# Autodesk Inventor assembly: Stewart_Platform
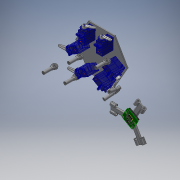
[picture p0: Inventor's stored thumbnail of the model, 180x180]
Saved by Autodesk Inventor 2019.4 (Build 234330000, 330)
## iProperties
Created: 2020-04-07
Part Number: Stewart_Platform
Document SubType Name: Assembly
Designer: Jorian Brusind
Author: Jorian Brusind
## Documents named in this file (7)
- C:\Users\Jorian Brusind\Documents\GitHub\PersonalProjects\Stewart Platform\Inventor Models\Stewart_Platform.iam
- C:\Users\Jorian Brusind\Documents\GitHub\PersonalProjects\Stewart Platform\Inventor Models\Top_.ipt
- C:\Users\Jorian Brusind\Documents\GitHub\PersonalProjects\Stewart Platform\Inventor Models\raspberry-pi-camera-module-v2-1.snapshot.3\RspCameraMia.iam
- C:\Users\Jorian Brusind\Documents\GitHub\PersonalProjects\Stewart Platform\Inventor Models\Bot_.ipt
- C:\Users\Jorian Brusind\Documents\GitHub\PersonalProjects\Stewart Platform\Inventor Models\tower-pro-sg90-micro-servo-2.snapshot.5\microservoAssembly.iam
- C:\Users\Jorian Brusind\Documents\GitHub\PersonalProjects\Stewart Platform\Inventor Models\tower-pro-sg90-micro-servo-2.snapshot.5\microservoArm.ipt
- C:\Users\Jorian Brusind\Documents\GitHub\PersonalProjects\Stewart Platform\Inventor Models\59935K140_METRIC BALL JOINT ROD END.ipt
## Components (21 placed, 6 different names)
1. Top_:1 — Mate:1, Mate:2, Mate:3
2. RspCameraMia:1 [sub-assembly] — Mate:1, Mate:2, Mate:3
3. Bot_:1 — Mate:4, Mate:5, Mate:6, Mate:7, Mate:8, Mate:9, Mate:10, Mate:11, Mate:12, Mate:13, Mate:14, Mate:15, Mate:16, Mate:17, Mate:18, Mate:19, Mate:20, Mate:21
4. microservoAssembly:1 [sub-assembly] — Mate:4, Mate:5, Mate:6, Mate:24, Mate:25
5. microservoAssembly:2 [sub-assembly] — Mate:8, Mate:9, Mate:10, Mate:22, Mate:23
6. microservoAssembly:3 [sub-assembly] — Mate:16, Mate:18, Mate:19, Mate:26, Mate:33
7. microservoAssembly:4 [sub-assembly] — Mate:11, Mate:12, Mate:13, Mate:29, Mate:31
8. microservoAssembly:5 [sub-assembly] — Mate:7, Mate:14, Mate:15, Mate:28, Mate:30
9. microservoAssembly:6 [sub-assembly] — Mate:17, Mate:20, Mate:21, Mate:27, Mate:32
10. microservoArm:1 — Mate:22, Mate:23
11. microservoArm:2 — Mate:24, Mate:25
12. microservoArm:3 — Mate:26, Mate:33, Mate:34, Mate:35
13. microservoArm:4 — Mate:28, Mate:30
14. microservoArm:5 — Mate:27, Mate:32, Mate:36, Mate:37
15. microservoArm:6 — Mate:29, Mate:31
16. 59935K140_METRIC BALL JOINT ROD END:1 — Mate:34, Mate:35
17. 59935K140_METRIC BALL JOINT ROD END:2 — Mate:36, Mate:37
18. 59935K140_METRIC BALL JOINT ROD END:3
19. 59935K140_METRIC BALL JOINT ROD END:4
20. 59935K140_METRIC BALL JOINT ROD END:5
21. 59935K140_METRIC BALL JOINT ROD END:6
## Relationships (37: Mate 37)
- Mate:1: Top_:1 ↔ RspCameraMia:1
- Mate:2: Top_:1 ↔ RspCameraMia:1
- Mate:3: Top_:1 ↔ RspCameraMia:1
- Mate:4: Bot_:1 ↔ microservoAssembly:1
- Mate:5 (0.3 mm): Bot_:1 ↔ microservoAssembly:1
- Mate:6 (0.2 mm): Bot_:1 ↔ microservoAssembly:1
- Mate:7: Bot_:1 ↔ microservoAssembly:5
- Mate:8: Bot_:1 ↔ microservoAssembly:2
- Mate:9 (0.3 mm): Bot_:1 ↔ microservoAssembly:2
- Mate:10 (0.2 mm): Bot_:1 ↔ microservoAssembly:2
- Mate:11: Bot_:1 ↔ microservoAssembly:4
- Mate:12 (0.3 mm): Bot_:1 ↔ microservoAssembly:4
- Mate:13 (0.2 mm): Bot_:1 ↔ microservoAssembly:4
- Mate:14 (0.3 mm): Bot_:1 ↔ microservoAssembly:5
- Mate:15 (0.2 mm): Bot_:1 ↔ microservoAssembly:5
- Mate:16: Bot_:1 ↔ microservoAssembly:3
- Mate:17: Bot_:1 ↔ microservoAssembly:6
- Mate:18 (0.3 mm): Bot_:1 ↔ microservoAssembly:3
- Mate:19 (0.2 mm): Bot_:1 ↔ microservoAssembly:3
- Mate:20 (0.3 mm): Bot_:1 ↔ microservoAssembly:6
- Mate:21 (0.2 mm): Bot_:1 ↔ microservoAssembly:6
- Mate:22: microservoAssembly:2 ↔ microservoArm:1
- Mate:23: microservoAssembly:2 ↔ microservoArm:1
- Mate:24: microservoAssembly:1 ↔ microservoArm:2
- Mate:25: microservoAssembly:1 ↔ microservoArm:2
- Mate:26: microservoAssembly:3 ↔ microservoArm:3
- Mate:27: microservoAssembly:6 ↔ microservoArm:5
- Mate:28: microservoAssembly:5 ↔ microservoArm:4
- Mate:29: microservoAssembly:4 ↔ microservoArm:6
- Mate:30: microservoAssembly:5 ↔ microservoArm:4
- Mate:31: microservoAssembly:4 ↔ microservoArm:6
- Mate:32: microservoAssembly:6 ↔ microservoArm:5
- Mate:33: microservoAssembly:3 ↔ microservoArm:3
- Mate:34: microservoArm:3 ↔ 59935K140_METRIC BALL JOINT ROD END:1
- Mate:35 (5 mm): microservoArm:3 ↔ 59935K140_METRIC BALL JOINT ROD END:1
- Mate:36: microservoArm:5 ↔ 59935K140_METRIC BALL JOINT ROD END:2
- Mate:37 (5 mm): microservoArm:5 ↔ 59935K140_METRIC BALL JOINT ROD END:2
